# Autodesk Inventor assembly: Ensamble
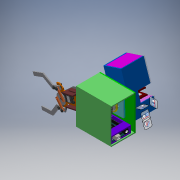
[picture p0: Inventor's stored thumbnail of the model, 180x180]
Saved by Autodesk Inventor 2019 (Build 230136000, 136)
## iProperties
Created: 2020-02-05
Part Number: Ensamble
Document SubType Name: Assembly
Designer: Omar
Author: Omar
## Documents named in this file (33)
- C:\Users\Silvia\Documents\Omar\BrazoRobotico\SERVOS\Diseño\Ensamble.iam
- C:\Users\Silvia\Documents\Omar\BrazoRobotico\SERVOS\Diseño\PIEZAS\Base_servo1.ipt
- C:\Users\Silvia\Documents\Omar\BrazoRobotico\SERVOS\Diseño\PIEZAS\Arduino.ipt
- C:\Users\Silvia\Documents\Omar\BrazoRobotico\SERVOS\Diseño\PIEZAS\Base_caja.ipt
- C:\Users\Silvia\Documents\Omar\BrazoRobotico\SERVOS\Diseño\PIEZAS\Servo HS-225MG\01.ipt
- C:\Users\Silvia\Documents\Omar\BrazoRobotico\SERVOS\Diseño\Libreria\en-US\GB_T 276-94 60000-Z\Bearing 6000-Z GB_T 276-94.ipt
- C:\Users\Silvia\Documents\Omar\BrazoRobotico\SERVOS\Diseño\PIEZAS\Base_tapa.ipt
- C:\Users\Silvia\Documents\Omar\BrazoRobotico\SERVOS\Diseño\PIEZAS\Base_giratorio.ipt
- C:\Users\Silvia\Documents\Omar\BrazoRobotico\SERVOS\Diseño\PIEZAS\MiniBreadboard.ipt
- C:\Users\Silvia\Documents\Omar\BrazoRobotico\SERVOS\Diseño\PIEZAS\Base_Arduino.ipt
- C:\Users\Silvia\Documents\Omar\BrazoRobotico\SERVOS\Diseño\PIEZAS\Base_sostenedor.ipt
- C:\Users\Silvia\Documents\Omar\BrazoRobotico\SERVOS\Diseño\PIEZAS\Base sostenedor1.ipt
- C:\Users\Silvia\Documents\Omar\BrazoRobotico\SERVOS\Diseño\PIEZAS\Pinza_sostenedor.ipt
- C:\Users\Silvia\Documents\Omar\BrazoRobotico\SERVOS\Diseño\PIEZAS\Pinza_dedo.ipt
- C:\Users\Silvia\Documents\Omar\BrazoRobotico\SERVOS\Diseño\PIEZAS\Giroservo.ipt
- C:\Users\Silvia\Documents\Omar\BrazoRobotico\SERVOS\Diseño\PIEZAS\Pinza_acople.ipt
- C:\Users\Silvia\Documents\Omar\BrazoRobotico\SERVOS\Diseño\Libreria\en-US\BS 290 SKF(21)\BS 290 SKF - SKF 626-RS1.ipt
- C:\Users\Silvia\Documents\Omar\BrazoRobotico\SERVOS\Diseño\Ensamble\Design Accelerator\Tornillo_servo.iam
- C:\Users\Silvia\Documents\Omar\BrazoRobotico\SERVOS\Diseño\Ensamble\Design Accelerator\Tornillos_pinza1.iam
- C:\Users\Silvia\Documents\Omar\BrazoRobotico\SERVOS\Diseño\Ensamble\Design Accelerator\Tornillos_pinza2.iam
- C:\Users\Silvia\Documents\Omar\BrazoRobotico\SERVOS\Diseño\Ensamble\Design Accelerator\Tornillos_pinza3.iam
- C:\Users\Silvia\Documents\Omar\BrazoRobotico\SERVOS\Diseño\Ensamble\Design Accelerator\Tornillos_pinza4.iam
- C:\Users\Silvia\Documents\Omar\BrazoRobotico\SERVOS\Diseño\PIEZAS\Hombro_servo.ipt
- C:\Users\Silvia\Documents\Omar\BrazoRobotico\SERVOS\Diseño\PIEZAS\Hombro_sostenedorcojin.ipt
- C:\Users\Silvia\Documents\Omar\BrazoRobotico\SERVOS\Diseño\PIEZAS\Eje.ipt
- C:\Users\Silvia\Documents\Omar\BrazoRobotico\SERVOS\Diseño\PIEZAS\Hombro_tapas.ipt
- C:\Users\Silvia\Documents\Omar\BrazoRobotico\SERVOS\Diseño\PIEZAS\Hombro_base.ipt
- C:\Users\Silvia\Documents\Omar\BrazoRobotico\SERVOS\Diseño\PIEZAS\Brazo_Inferior.ipt
- C:\Users\Silvia\Documents\Omar\BrazoRobotico\SERVOS\Diseño\PIEZAS\Brazo_union.ipt
- C:\Users\Silvia\Documents\Omar\BrazoRobotico\SERVOS\Diseño\PIEZAS\Brazo_eje.ipt
- C:\Users\Silvia\Documents\Omar\BrazoRobotico\SERVOS\Diseño\PIEZAS\Brazo_Superior.ipt
- C:\Users\Silvia\Documents\Omar\BrazoRobotico\SERVOS\Diseño\PIEZAS\Hombro_tapag.ipt
- C:\Users\Silvia\Documents\Omar\BrazoRobotico\SERVOS\Diseño\PIEZAS\Hombro_tapapeq.ipt
## Components (46 placed, 32 different names)
1. Base_servo1:1 — Mate:7, Mate:8, Mate:14, Flush:7, Mate:103
2. Arduino:1 — Mate:18, Mate:19, Mate:20
3. Base_caja:1 — Mate:1, Mate:3, Mate:4, Mate:14, Flush:7, Mate:21, Mate:22, Flush:8, Flush:31, Flush:32, Flush:33, Mate:104
4. 01:1 — Mate:7, Mate:8, Mate:9, Mate:10
5. Rolling bearing GB/T 276-1994 Type 60000-Z 6000-Z:1 — Mate:5, Mate:11, Mate:12, Mate:26
6. Base_tapa:1 — Mate:4, Mate:5, Mate:82, Flush:31, Flush:32
7. Base_giratorio:1 — Mate:9, Mate:10, Mate:11, Mate:12, Mate:23, Mate:27, Mate:80, Mate:81, Rotation:1
8. MiniBreadboard:1 — Mate:103, Flush:33, Mate:104
9. Base_Arduino:1 — Mate:18, Mate:19, Mate:20, Mate:21, Mate:22, Flush:8
10. Base_sostenedor:1 — Mate:23, Mate:26, Mate:29
11. Base sostenedor1:2 — Mate:27, Mate:29, Mate:82
12. 01:2 — Mate:33, Flush:11, Mate:34, Mate:35, Mate:36
13. Giroservo:1 — Mate:33, Flush:11, Mate:38, Mate:39, Mate:43, Mate:44
14. Pinza_sostenedor:1 — Mate:34, Mate:35, Mate:36, Mate:37, Mate:42, Mate:47, Mate:48, Mate:83, Mate:84, Mate:85, Mate:100
15. Pinza_dedo:1 — Mate:37, Mate:40, Mate:41, Mate:49, Mate:50
16. Pinza_dedo:2 — Mate:42, Mate:45, Mate:46, Mate:51, Mate:52
17. Pinza_acople:1 — Mate:38, Mate:39, Mate:40, Mate:41, Mate:55, Mate:56
18. Pinza_acople:2 — Mate:43, Mate:44, Mate:45, Mate:46, Mate:53, Mate:54
19. BS 290 SKF- with RS1 seal SKF 626-RS1:1 — Mate:57, Flush:12, Mate:68
20. Tornillos_servo:1 [sub-assembly] — Mate:47, Mate:48, Mate:100
21. Tornillos_pinza1:1 [sub-assembly] — Mate:49, Mate:50
22. Tornillos_pinza2:1 [sub-assembly] — Mate:51, Mate:52
23. Tornillos_pinza3:1 [sub-assembly] — Mate:53, Mate:54
24. Tornillos_pinza4:1 [sub-assembly] — Mate:55, Mate:56
25. Hombro_servo:1 — Mate:63, Mate:64, Mate:65, Angle:1, Mate:71, Flush:18, Flush:19, Mate:77
26. Hombro_sostenedorcojin:1 — Mate:57, Flush:12, Angle:1, Mate:71, Angle:2, Mate:74, Flush:36
27. 01:3 — Mate:58, Flush:13, Mate:63, Mate:64, Mate:65
28. Giroservo:2 — Mate:58, Flush:13, Mate:66, Mate:67
29. Eje:1 — Mate:66, Mate:67, Mate:68, Mate:72, Mate:73, Mate:127, Mate:129
30. BS 290 SKF- with RS1 seal SKF 626-RS1:2 — Mate:73
31. Hombro_sostenedorcojin:2 — Angle:3, Mate:75, Angle:4, Flush:16, Flush:17, Mate:76
32. BS 290 SKF- with RS1 seal SKF 626-RS1:3 — Mate:72
33. Hombro_sostenedorcojin:3 — Angle:2, Angle:3, Mate:74, Mate:75
34. Hombro_tapas:1 — Angle:4, Flush:16, Flush:17, Mate:76, Flush:40
35. Hombro_tapas:2 — Flush:18, Flush:19, Mate:77, Flush:20, Mate:78, Mate:79, Flush:37
36. Hombro_base:1 — Flush:20, Mate:78, Mate:79, Mate:80, Mate:81, Rotation:1, Flush:38, Mate:130, Flush:39, Mate:131
37. Brazo_Inferior:1 — Flush:22, Mate:83, Mate:84, Mate:85, Flush:23, Flush:24, Mate:86, Flush:25, Mate:87, Mate:88, Flush:26, Mate:89, Mate:90, Mate:124
38. Brazo_Inferior:2 — Flush:22, Flush:23, Flush:24, Mate:86, Mate:123
39. Brazo_union:1 — Flush:25, Mate:87, Mate:88, Mate:119, Mate:120, Mate:121, Mate:122
40. Brazo_union:2 — Flush:26, Mate:89, Mate:90
41. Brazo_Superior:1 — Mate:119, Mate:120, Mate:123, Mate:128, Flush:35
42. Brazo_Superior:2 — Mate:121, Mate:122, Mate:124, Mate:125, Mate:126, Flush:34, Flush:36
43. Brazo_eje:2 — Mate:125, Mate:126, Mate:127, Flush:34
44. Brazo_eje:3 — Mate:128, Mate:129, Flush:35
45. Hombro_tapag:1 — Flush:37, Flush:38, Mate:130
46. Hombro_tapapeq:1 — Flush:39, Flush:40, Mate:131
## Relationships (122: Mate 90, Flush 27, Angle 4, RelateRotation 1)
- Mate:1: Base_caja:1
- Mate:3: Base_caja:1
- Mate:4: Base_caja:1 ↔ Base_tapa:1
- Mate:5: Rolling bearing GB/T 276-1994 Type 60000-Z 6000-Z:1 ↔ Base_tapa:1
- Mate:7: Base_servo1:1 ↔ 01:1
- Mate:8: Base_servo1:1 ↔ 01:1
- Mate:9: 01:1 ↔ Base_giratorio:1
- Mate:10: 01:1 ↔ Base_giratorio:1
- Mate:11: Rolling bearing GB/T 276-1994 Type 60000-Z 6000-Z:1 ↔ Base_giratorio:1
- Mate:12: Rolling bearing GB/T 276-1994 Type 60000-Z 6000-Z:1 ↔ Base_giratorio:1
- Mate:14: Base_servo1:1 ↔ Base_caja:1
- Flush:7: Base_servo1:1 ↔ Base_caja:1
- Mate:18: Arduino:1 ↔ Base_Arduino:1
- Mate:19: Arduino:1 ↔ Base_Arduino:1
- Mate:20: Arduino:1 ↔ Base_Arduino:1
- Mate:21: Base_caja:1 ↔ Base_Arduino:1
- Mate:22: Base_caja:1 ↔ Base_Arduino:1
- Flush:8: Base_caja:1 ↔ Base_Arduino:1
- Mate:23: Base_giratorio:1 ↔ Base_sostenedor:1
- Mate:26: Rolling bearing GB/T 276-1994 Type 60000-Z 6000-Z:1 ↔ Base_sostenedor:1
- Mate:27: Base_giratorio:1 ↔ Base sostenedor1:2
- Mate:29: Base_sostenedor:1 ↔ Base sostenedor1:2
- Mate:33: 01:2 ↔ Giroservo:1
- Flush:11 (1 mm): 01:2 ↔ Giroservo:1
- Mate:34: 01:2 ↔ Pinza_sostenedor:1
- Mate:35 (0.152 mm): 01:2 ↔ Pinza_sostenedor:1
- Mate:36 (2 mm): 01:2 ↔ Pinza_sostenedor:1
- Mate:37: Pinza_sostenedor:1 ↔ Pinza_dedo:1
- Mate:38: Giroservo:1 ↔ Pinza_acople:1
- Mate:39: Giroservo:1 ↔ Pinza_acople:1
- Mate:40: Pinza_dedo:1 ↔ Pinza_acople:1
- Mate:41: Pinza_dedo:1 ↔ Pinza_acople:1
- Mate:42: Pinza_sostenedor:1 ↔ Pinza_dedo:2
- Mate:43: Giroservo:1 ↔ Pinza_acople:2
- Mate:44: Giroservo:1 ↔ Pinza_acople:2
- Mate:45: Pinza_dedo:2 ↔ Pinza_acople:2
- Mate:46: Pinza_dedo:2 ↔ Pinza_acople:2
- Mate:47: Pinza_sostenedor:1 ↔ Tornillos_servo:1
- Mate:48: Pinza_sostenedor:1 ↔ Tornillos_servo:1
- Mate:49: Pinza_dedo:1 ↔ Tornillos_pinza1:1
- Mate:50: Pinza_dedo:1 ↔ Tornillos_pinza1:1
- Mate:51: Pinza_dedo:2 ↔ Tornillos_pinza2:1
- Mate:52: Pinza_dedo:2 ↔ Tornillos_pinza2:1
- Mate:53: Pinza_acople:2 ↔ Tornillos_pinza3:1
- Mate:54: Pinza_acople:2 ↔ Tornillos_pinza3:1
- Mate:55: Pinza_acople:1 ↔ Tornillos_pinza4:1
- Mate:56: Pinza_acople:1 ↔ Tornillos_pinza4:1
- Mate:57: BS 290 SKF- with RS1 seal SKF 626-RS1:1 ↔ Hombro_sostenedorcojin:1
- Flush:12 (1.5 mm): BS 290 SKF- with RS1 seal SKF 626-RS1:1 ↔ Hombro_sostenedorcojin:1
- Mate:58: 01:3 ↔ Giroservo:2
- Flush:13 (1 mm): 01:3 ↔ Giroservo:2
- Mate:63 (1.618 mm): Hombro_servo:1 ↔ 01:3
- Mate:64 (2 mm): Hombro_servo:1 ↔ 01:3
- Mate:65: Hombro_servo:1 ↔ 01:3
- Mate:66: Giroservo:2 ↔ Eje:1
- Mate:67: Giroservo:2 ↔ Eje:1
- Mate:68: BS 290 SKF- with RS1 seal SKF 626-RS1:1 ↔ Eje:1
- [Mate]: BS 290 SKF- with RS1 seal SKF 626-RS1:2 ↔ Hombro_sostenedorcojin:2
- [Flush] (1.5 mm): BS 290 SKF- with RS1 seal SKF 626-RS1:2 ↔ Hombro_sostenedorcojin:2
- [Mate]: BS 290 SKF- with RS1 seal SKF 626-RS1:3 ↔ Hombro_sostenedorcojin:3
- [Flush] (1.5 mm): BS 290 SKF- with RS1 seal SKF 626-RS1:3 ↔ Hombro_sostenedorcojin:3
- Angle:1 (0 deg): Hombro_servo:1 ↔ Hombro_sostenedorcojin:1
- Mate:71 (20 mm): Hombro_servo:1 ↔ Hombro_sostenedorcojin:1
- Mate:72: Eje:1 ↔ BS 290 SKF- with RS1 seal SKF 626-RS1:3
- Mate:73: Eje:1 ↔ BS 290 SKF- with RS1 seal SKF 626-RS1:2
- Angle:2 (0 deg): Hombro_sostenedorcojin:1 ↔ Hombro_sostenedorcojin:3
- Angle:3 (0 deg): Hombro_sostenedorcojin:2 ↔ Hombro_sostenedorcojin:3
- Mate:74 (30 mm): Hombro_sostenedorcojin:1 ↔ Hombro_sostenedorcojin:3
- Mate:75 (5 mm): Hombro_sostenedorcojin:2 ↔ Hombro_sostenedorcojin:3
- Angle:4 (0 deg): Hombro_sostenedorcojin:2 ↔ Hombro_tapas:1
- Flush:16: Hombro_sostenedorcojin:2 ↔ Hombro_tapas:1
- Flush:17: Hombro_sostenedorcojin:2 ↔ Hombro_tapas:1
- Mate:76 (15 mm): Hombro_sostenedorcojin:2 ↔ Hombro_tapas:1
- Flush:18: Hombro_servo:1 ↔ Hombro_tapas:2
- Flush:19: Hombro_servo:1 ↔ Hombro_tapas:2
- Mate:77 (35 mm): Hombro_servo:1 ↔ Hombro_tapas:2
- Flush:20: Hombro_tapas:2 ↔ Hombro_base:1
- Mate:78: Hombro_tapas:2 ↔ Hombro_base:1
- Mate:79: Hombro_tapas:2 ↔ Hombro_base:1
- Mate:80: Base_giratorio:1 ↔ Hombro_base:1
- Mate:81: Base_giratorio:1 ↔ Hombro_base:1
- Rotation:1 [RelateRotation] (9 ul): Base_giratorio:1 ↔ Hombro_base:1
- Mate:82: Base_tapa:1 ↔ Base sostenedor1:2
- Flush:22: Brazo_Inferior:1 ↔ Brazo_Inferior:2
- Mate:83: Pinza_sostenedor:1 ↔ Brazo_Inferior:1
- Mate:84: Pinza_sostenedor:1 ↔ Brazo_Inferior:1
- Mate:85: Pinza_sostenedor:1 ↔ Brazo_Inferior:1
- Flush:23: Brazo_Inferior:1 ↔ Brazo_Inferior:2
- Flush:24: Brazo_Inferior:1 ↔ Brazo_Inferior:2
- Mate:86 (30 mm): Brazo_Inferior:1 ↔ Brazo_Inferior:2
- Flush:25 (2 mm): Brazo_Inferior:1 ↔ Brazo_union:1
- Mate:87: Brazo_Inferior:1 ↔ Brazo_union:1
- Mate:88: Brazo_Inferior:1 ↔ Brazo_union:1
- Flush:26 (-2 mm): Brazo_Inferior:1 ↔ Brazo_union:2
- Mate:89: Brazo_Inferior:1 ↔ Brazo_union:2
- Mate:90: Brazo_Inferior:1 ↔ Brazo_union:2
- Mate:100: Pinza_sostenedor:1 ↔ Tornillos_servo:1
- Flush:31: Base_caja:1 ↔ Base_tapa:1
- Flush:32: Base_caja:1 ↔ Base_tapa:1
- Mate:103 (1 mm): Base_servo1:1 ↔ MiniBreadboard:1
- Flush:33 (20 mm): Base_caja:1 ↔ MiniBreadboard:1
- Mate:104: Base_caja:1 ↔ MiniBreadboard:1
- Mate:119: Brazo_union:1 ↔ Brazo_Superior:1
- Mate:120: Brazo_union:1 ↔ Brazo_Superior:1
- Mate:121: Brazo_union:1 ↔ Brazo_Superior:2
- Mate:122: Brazo_union:1 ↔ Brazo_Superior:2
- Mate:123 (5 mm): Brazo_Inferior:2 ↔ Brazo_Superior:1
- Mate:124 (5 mm): Brazo_Inferior:1 ↔ Brazo_Superior:2
- Mate:125: Brazo_Superior:2 ↔ Brazo_eje:2
- Mate:126: Brazo_Superior:2 ↔ Brazo_eje:2
- Mate:127: Eje:1 ↔ Brazo_eje:2
- Flush:34 (-2 mm): Brazo_Superior:2 ↔ Brazo_eje:2
- Mate:128: Brazo_Superior:1 ↔ Brazo_eje:3
- Mate:129: Eje:1 ↔ Brazo_eje:3
- Flush:35 (2 mm): Brazo_Superior:1 ↔ Brazo_eje:3
- Flush:36 (8 mm): Hombro_sostenedorcojin:1 ↔ Brazo_Superior:2
- Flush:37: Hombro_tapas:2 ↔ Hombro_tapag:1
- Flush:38: Hombro_base:1 ↔ Hombro_tapag:1
- Mate:130: Hombro_base:1 ↔ Hombro_tapag:1
- Flush:39: Hombro_base:1 ↔ Hombro_tapapeq:1
- Flush:40: Hombro_tapas:1 ↔ Hombro_tapapeq:1
- Mate:131: Hombro_base:1 ↔ Hombro_tapapeq:1
## Named parameters: d116_d100 = 0 mm, d117_d101 = 1.5 mm, d118_d100 = 0 mm, d119_d101 = 1.5 mm
